# Autodesk Inventor assembly: stilladssøjle
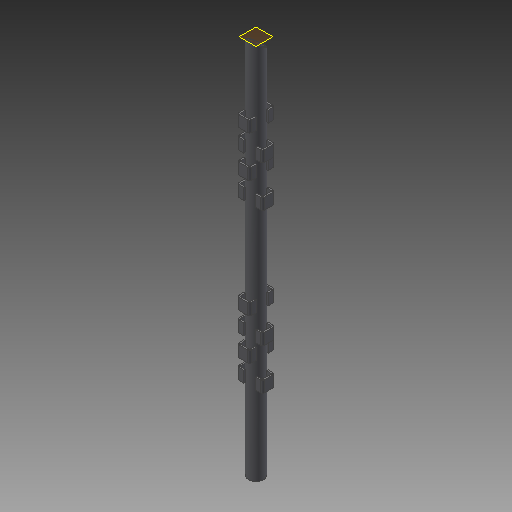
[picture p0: Inventor's stored thumbnail of the model, 512x512]
Saved by Autodesk Inventor 2018 (Build 220112000, 112)
## iProperties
Created: 2019-09-25
Part Number: stilladssøjle
Document SubType Name: Assembly
Designer: loppen
Mass: 6435.91 g
Surface Area: 4290.18 cm^2
Volume: 819.862 cm^3
Density: 7.85 g/cm^3
Author: loppen
## Documents named in this file (3)
- Z:\trappe\baluster\stilladssøjle.iam
- Z:\trappe\baluster\rør.ipt
- Z:\trappe\baluster\øre.ipt
## Components (17 placed, 2 different names)
1. rør:1 — Mate:1, Tangent:1, Mate:2, Tangent:2, Flush:2, Flush:7, Flush:8, Tangent:3, Tangent:4, Flush:11, Flush:12, Tangent:5, Tangent:6, Tangent:7, Mate:3, Mate:4, Tangent:8
2. øre:6 — Flush:12, Tangent:5, Flush:13, Flush:15
3. øre:1 — Mate:1, Tangent:1, Flush:1, Flush:2, Flush:9, Flush:17
4. øre:2 — Mate:2, Tangent:2, Flush:1, Flush:10
5. øre:3 — Flush:7, Tangent:3, Flush:9
6. øre:4 — Flush:8, Tangent:4, Flush:10
7. øre:5 — Flush:11, Tangent:6, Flush:13, Flush:16, Flush:17
8. øre:7 — Tangent:7, Mate:3, Flush:16
9. øre:8 — Tangent:8, Mate:4, Flush:15
10. øre:9
11. øre:10
12. øre:11
13. øre:12
14. øre:13
15. øre:14
16. øre:15
17. øre:16
## Component patterns: (2 elements, first: øre:6 + øre:1 + øre:2 + øre:3 + øre:4 + øre:5 + øre:7 + øre:8)
## Relationships (26: Flush 14, Tangent 8, Mate 4)
- Mate:1: rør:1 ↔ øre:1
- Tangent:1: rør:1 ↔ øre:1
- Mate:2: rør:1 ↔ øre:2
- Tangent:2: rør:1 ↔ øre:2
- Flush:1 (-130 mm): øre:1 ↔ øre:2
- Flush:2 (-200 mm): rør:1 ↔ øre:1
- [Flush] (-130 mm): øre:3 ↔ øre:4
- Flush:7: rør:1 ↔ øre:3
- Flush:8: rør:1 ↔ øre:4
- Tangent:3: rør:1 ↔ øre:3
- Tangent:4: rør:1 ↔ øre:4
- Flush:9: øre:1 ↔ øre:3
- Flush:10: øre:2 ↔ øre:4
- Flush:11: rør:1 ↔ øre:5
- Flush:12: rør:1 ↔ øre:6
- Tangent:5: rør:1 ↔ øre:6
- Tangent:6: rør:1 ↔ øre:5
- Flush:13 (-130 mm): øre:6 ↔ øre:5
- [Flush] (-130 mm): øre:7 ↔ øre:8
- Tangent:8: rør:1 ↔ øre:8
- Tangent:7: rør:1 ↔ øre:7
- Mate:3: rør:1 ↔ øre:7
- Mate:4: rør:1 ↔ øre:8
- Flush:15: øre:6 ↔ øre:8
- Flush:16: øre:5 ↔ øre:7
- Flush:17 (-82 mm): øre:1 ↔ øre:5
